# Autodesk Inventor assembly: STM32F103C8T6_Blue_Pill v6
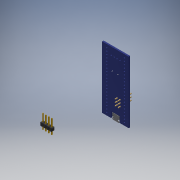
[picture p0: Inventor's stored thumbnail of the model, 180x180]
Saved by Autodesk Inventor 2018 (Build 220112000, 112)
## iProperties
Created: 2017-12-31
Part Number: STM32F103C8T6_Blue_Pill v6
Document SubType Name: Assembly
Designer: ZEUSLAP
Sending System: Autodesk Translation Framework v6.5.0.72
Preprocessor: ST-DEVELOPER v16.13
Title: C:/Users/Oresama/Dropbox/hobby/STM32F103C8/3D_Model/STM32F103C8T6_Blue_Pill v6.step
Author: denshikousakusenka
## Documents named in this file (9)
- C:\Users\ZEUSLAP\YandexDisk\Inventor\comparative_air_pollution_sensor\module_ppd42\parts\STM32F103C8T6_Blue_Pill v6\STM32F103C8T6_Blue_Pill v6.iam
- C:\Users\ZEUSLAP\YandexDisk\Inventor\comparative_air_pollution_sensor\module_ppd42\parts\STM32F103C8T6_Blue_Pill v6\Oscillator_HC-49_S v1.ipt
- C:\Users\ZEUSLAP\YandexDisk\Inventor\comparative_air_pollution_sensor\module_ppd42\parts\STM32F103C8T6_Blue_Pill v6\STM32F103C8T6_BluePill_Board v6.ipt
- C:\Users\ZEUSLAP\YandexDisk\Inventor\comparative_air_pollution_sensor\module_ppd42\parts\STM32F103C8T6_Blue_Pill v6\Oscillator_MC-306 v3.ipt
- C:\Users\ZEUSLAP\YandexDisk\Inventor\comparative_air_pollution_sensor\module_ppd42\parts\STM32F103C8T6_Blue_Pill v6\STM32_LQFP48 v3.ipt
- C:\Users\ZEUSLAP\YandexDisk\Inventor\comparative_air_pollution_sensor\module_ppd42\parts\STM32F103C8T6_Blue_Pill v6\Tactile_SMD_5x5mm v1.ipt
- C:\Users\ZEUSLAP\YandexDisk\Inventor\comparative_air_pollution_sensor\module_ppd42\parts\STM32F103C8T6_Blue_Pill v6\micro_usb_socket v1.ipt
- C:\Users\ZEUSLAP\YandexDisk\Inventor\comparative_air_pollution_sensor\module_ppd42\parts\STM32F103C8T6_Blue_Pill v6\Header_Male_2x3x11.6 v2.ipt
- C:\Users\ZEUSLAP\YandexDisk\Inventor\comparative_air_pollution_sensor\module_ppd42\parts\STM32F103C8T6_Blue_Pill v6\Pin Header 1x4 TH Pitch 2.54mm.ipt
## Components (8 placed, 8 different names)
1. Oscillator_HC-49/S v1:1
2. STM32F103C8T6_BluePill_Board v6:1 — Mate:1, Angle:1
3. Oscillator_MC-306 v3:1
4. STM32_LQFP48 v3:1
5. Tactile_SMD_5x5mm v1:1
6. micro_usb_socket v1:1
7. Header_Male_2x3x11.6 v2:1
8. Pin Header 1x4 TH Pitch 2.54mm:1 — Mate:1, Angle:1
## Relationships (2: Mate 1, Angle 1)
- Mate:1: STM32F103C8T6_BluePill_Board v6:1 ↔ Pin Header 1x4 TH Pitch 2.54mm:1
- Angle:1 (0 deg): STM32F103C8T6_BluePill_Board v6:1 ↔ Pin Header 1x4 TH Pitch 2.54mm:1
